# Autodesk Inventor assembly: Turntable-ArmConnection
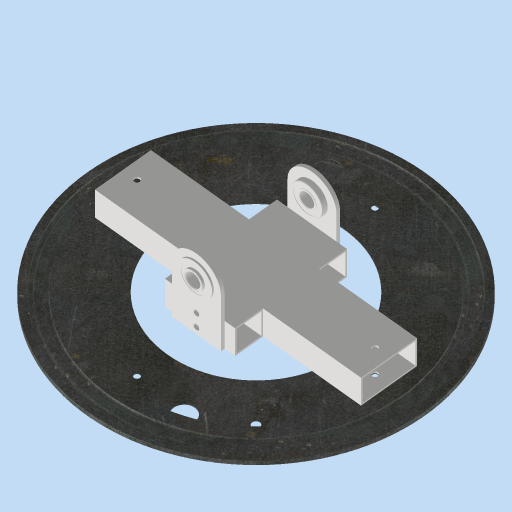
[picture p0: Inventor's stored thumbnail of the model, 512x512]
Saved by Autodesk Inventor 2024 (Build 280153000, 153)
## iProperties
Created: 2024-01-10
Part Number: Turntable-ArmConnection
Document SubType Name: Assembly
Designer: megan
Author: megan
## Documents named in this file (6)
- C:\Users\megan\OneDrive\Documents\GitHub\BehrendURCMechanical\CAD\Apparatus\Arm Base\Turntable-ArmConnection.iam
- C:\Users\megan\OneDrive\Documents\GitHub\BehrendURCMechanical\CAD\Apparatus\Arm Base\1544T3_Lubricated Turntable.ipt
- C:\Users\megan\OneDrive\Documents\GitHub\BehrendURCMechanical\CAD\Apparatus\Arm Base\2inTubeBase.ipt
- C:\Users\megan\OneDrive\Documents\GitHub\BehrendURCMechanical\CAD\Apparatus\Arm Base\1inTubeBase.ipt
- C:\Users\megan\OneDrive\Documents\GitHub\BehrendURCMechanical\CAD\Apparatus\Arm Base\ArmPlateBase.ipt
- C:\Users\megan\Downloads\6384K361_Ball Bearing\6384K361_Ball Bearing.ipt
## Components (8 placed, 5 different names)
1. 1544T3_Lubricated Turntable:1 — Mate:1, Mate:2, Mate:3
2. 2inTubeBase:1 — Mate:1, Mate:2, Mate:3, Mate:4, Mate:5, Mate:6, Mate:7, Mate:8, Mate:9
3. 1inTubeBase:1 — Mate:7, Mate:8, Mate:9, Mate:10, Mate:11, Mate:12
4. 1inTubeBase:2 — Mate:4, Mate:5, Mate:6, Mate:13, Mate:14, Mate:15
5. ArmPlateBase:1 — Mate:13, Mate:14, Mate:15, Mate:18, Mate:19
6. ArmPlateBase:2 — Mate:10, Mate:11, Mate:12, Mate:16, Mate:17
7. 6384K361_Ball Bearing:1 — Mate:16, Mate:17
8. 6384K361_Ball Bearing:2 — Mate:18, Mate:19
## Relationships (19: Mate 19)
- Mate:1: 1544T3_Lubricated Turntable:1 ↔ 2inTubeBase:1
- Mate:2: 1544T3_Lubricated Turntable:1 ↔ 2inTubeBase:1
- Mate:3: 1544T3_Lubricated Turntable:1 ↔ 2inTubeBase:1
- Mate:4: 2inTubeBase:1 ↔ 1inTubeBase:2
- Mate:5: 2inTubeBase:1 ↔ 1inTubeBase:2
- Mate:6: 2inTubeBase:1 ↔ 1inTubeBase:2
- Mate:7: 2inTubeBase:1 ↔ 1inTubeBase:1
- Mate:8: 2inTubeBase:1 ↔ 1inTubeBase:1
- Mate:9: 2inTubeBase:1 ↔ 1inTubeBase:1
- Mate:10: 1inTubeBase:1 ↔ ArmPlateBase:2
- Mate:11: 1inTubeBase:1 ↔ ArmPlateBase:2
- Mate:12: 1inTubeBase:1 ↔ ArmPlateBase:2
- Mate:13: 1inTubeBase:2 ↔ ArmPlateBase:1
- Mate:14: 1inTubeBase:2 ↔ ArmPlateBase:1
- Mate:15: 1inTubeBase:2 ↔ ArmPlateBase:1
- Mate:16: ArmPlateBase:2 ↔ 6384K361_Ball Bearing:1
- Mate:17: ArmPlateBase:2 ↔ 6384K361_Ball Bearing:1
- Mate:18: ArmPlateBase:1 ↔ 6384K361_Ball Bearing:2
- Mate:19: ArmPlateBase:1 ↔ 6384K361_Ball Bearing:2
